# Autodesk Inventor assembly: Synchronous Belts Transmission
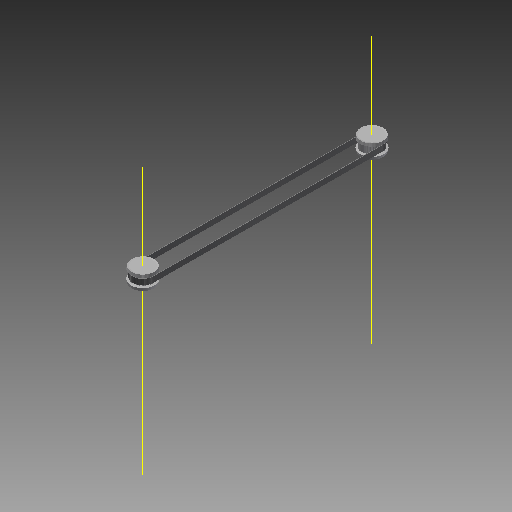
[picture p0: Inventor's stored thumbnail of the model, 512x512]
Saved by Autodesk Inventor 2017 SP1 (Build 210196100, 196)
## iProperties
Created: 2017-11-17
Part Number: Synchronous Belts Transmission
Document SubType Name: Assembly
Designer: Biscuit
ClientObjectVersion: 1
Author: Biscuit
## Documents named in this file (4)
- C:\Users\Cortman\Google Drive\ENSEIRB\EIRBOT\COUPE 2018\Cubes\assemblage\Design Accelerator\Synchronous Belts Transmission1.iam
- C:\Users\Cortman\Google Drive\ENSEIRB\EIRBOT\COUPE 2018\Cubes\assemblage\Design Accelerator\Synchronous Belt1.ipt
- C:\Users\Cortman\Google Drive\ENSEIRB\EIRBOT\COUPE 2018\Cubes\assemblage\Design Accelerator\Synchronous Pulley11.ipt
- C:\Users\Cortman\Google Drive\ENSEIRB\EIRBOT\COUPE 2018\Cubes\assemblage\Design Accelerator\Synchronous Pulley21.ipt
## Components (3 placed, 3 different names)
1. Synchronous Belt:1 — Affleurement:1, Placage:1, Placage:2, Affleurement:2, Placage:3, Placage:4
2. Synchronous Pulley1:1 — Affleurement:1, Placage:1, Placage:2, Rotation:1
3. Synchronous Pulley2:1 — Affleurement:2, Placage:3, Rotation:1, Placage:4
## Relationships (7: Mate 4, Flush 2, RelateRotation 1)
- Affleurement:1 [Flush]: Synchronous Belt:1 ↔ Synchronous Pulley1:1
- Placage:1 [Mate]: Synchronous Belt:1 ↔ Synchronous Pulley1:1
- Placage:2 [Mate]: Synchronous Belt:1 ↔ Synchronous Pulley1:1
- Affleurement:2 [Flush]: Synchronous Belt:1 ↔ Synchronous Pulley2:1
- Placage:3 [Mate]: Synchronous Belt:1 ↔ Synchronous Pulley2:1
- Rotation:1 [RelateRotation] (1 ul): Synchronous Pulley1:1 ↔ Synchronous Pulley2:1
- Placage:4 [Mate]: Synchronous Belt:1 ↔ Synchronous Pulley2:1
